# Autodesk Inventor assembly: LED-Board-Assembly
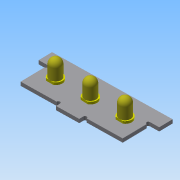
[picture p0: Inventor's stored thumbnail of the model, 180x180]
Saved by Autodesk Inventor 2016 (Build 200138000, 138)
## iProperties
Created: 2016-03-31
Part Number: LED-Board-Assembly
Document SubType Name: Assembly
Designer: admin
Author: admin
## Documents named in this file (3)
- E:\Alex\HS-Spectrophotometer\parts\New vesion\AK-C-C10-LED-Board-Assembly.iam
- E:\Alex\HS-Spectrophotometer\parts\New vesion\AK-C-C10-LED-Board.ipt
- E:\Alex\HS-Spectrophotometer\parts\Common\LED.ipt
## Components (4 placed, 2 different names)
1. AK-C-C10-LED-Board:1 — Mate:1, Mate:2, Mate:3, Mate:4, Mate:5, Mate:6
2. LED:1 — Mate:1, Mate:4
3. LED:2 — Mate:2, Mate:5
4. LED:3 — Mate:3, Mate:6
## Relationships (6: Mate 6)
- Mate:1: AK-C-C10-LED-Board:1 ↔ LED:1
- Mate:2: AK-C-C10-LED-Board:1 ↔ LED:2
- Mate:3: AK-C-C10-LED-Board:1 ↔ LED:3
- Mate:4: AK-C-C10-LED-Board:1 ↔ LED:1
- Mate:5: AK-C-C10-LED-Board:1 ↔ LED:2
- Mate:6: AK-C-C10-LED-Board:1 ↔ LED:3
